# Autodesk Inventor assembly: BrailleTyper
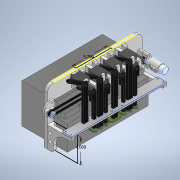
[picture p0: Inventor's stored thumbnail of the model, 180x180]
Saved by Autodesk Inventor 2020.1 (Build 241239000, 239)
## iProperties
Created: 2020-02-22
Part Number: BrailleTyper
Document SubType Name: Assembly
Designer: Dominic
Author: Dominic
## Documents named in this file (21)
- C:\Users\panzi\Dropbox\Projects\Braille\BrailleTyper.iam
- C:\Users\panzi\Dropbox\Projects\Braille\RoughMachine.ipt
- C:\Users\panzi\Dropbox\Projects\Braille\Servo.ipt
- C:\Users\panzi\Dropbox\Projects\Braille\KeyLever.ipt
- C:\Users\panzi\Dropbox\Projects\Braille\ShortBraillePlunger.ipt
- C:\Users\panzi\Dropbox\Projects\Braille\PlungerPlate.ipt
- C:\Users\panzi\Dropbox\Projects\Braille\LongBraillePlunger.ipt
- C:\Users\panzi\Dropbox\Projects\Braille\BigServo.ipt
- C:\Users\panzi\Dropbox\Projects\Braille\NewLinePlunger.ipt
- C:\Users\panzi\Dropbox\Projects\Braille\KeyLeverNewLine.ipt
- C:\Users\panzi\Dropbox\Projects\Braille\Pulley.ipt
- C:\Users\panzi\Dropbox\Projects\Braille\Belt.ipt
- C:\Users\panzi\Dropbox\Projects\Braille\Frame.ipt
- C:\Users\panzi\Dropbox\Projects\Braille\ServoMount.ipt
- C:\Users\panzi\Dropbox\Projects\Braille\ReturnFinger.ipt
- C:\Users\panzi\Dropbox\Projects\Braille\PlungerPlateBracket.ipt
- C:\Users\panzi\Dropbox\Projects\Braille\BigServoMount.ipt
- C:\Users\panzi\Dropbox\Projects\Braille\Tensioner.ipt
- C:\Users\panzi\Dropbox\Projects\Braille\ldo_motor_multiple_configs.ipt
- C:\Users\panzi\Dropbox\Projects\Braille\MotorMount.ipt
- C:\Users\panzi\Dropbox\Projects\Braille\PlungerPlateBracket_MIR1.ipt
## Components (44 placed, 20 different names)
1. RoughMachine:1 — Flush:8, Mate:16, Flush:21, Mate:25, Mate:54, Mate:61, Flush:28, Flush:29
2. Servo:2 — Flush:2, Flush:12, Mate:15, Flush:24, Mate:75, Mate:80, Mate:100, Mate:101, Mate:102
3. Servo:3 — Flush:2, Flush:3, Flush:11, Mate:6, Mate:13, Mate:69, Mate:70, Mate:71
4. Servo:4 — Flush:3, Flush:4, Flush:13, Mate:72, Mate:73, Mate:74, Mate:77, Mate:78
5. Servo:5 — Flush:4, Flush:5, Flush:10, Flush:11, Mate:4, Mate:12, Mate:91, Mate:92, Mate:93
6. Servo:6 — Flush:5, Flush:6, Flush:9, Flush:10, Mate:7, Mate:10, Mate:97, Mate:98, Mate:99
7. Servo:7 — Flush:6, Flush:7, Flush:9, Mate:1, Mate:8, Mate:15, Mate:16, Mate:103, Mate:104, Mate:105
8. Servo:8 — Flush:7, Flush:8, Flush:12, Flush:13, Mate:76, Mate:79, Mate:94, Mate:95, Mate:96
9. KeyLever:1 — Mate:1, Mate:8, Mate:128, Mate:129
10. KeyLever:4 — Mate:4, Mate:12, Mate:89, Mate:127
11. KeyLever:6 — Mate:6, Mate:13, Mate:28, Mate:90
12. KeyLever:7 — Mate:7, Mate:10, Mate:26, Mate:88
13. PlungerPlate:1 — Flush:21, Mate:25, Mate:32, Mate:33, Mate:34, Mate:42, Mate:43, Mate:44, Mate:53, Mate:109, Mate:110, Mate:111, Mate:125, Mate:126, Mate:130
14. ShortBraillePlunger:2 — Mate:26, Mate:32, Mate:88
15. ShortBraillePlunger:3 — Mate:33, Mate:89, Mate:126, Mate:127
16. ShortBraillePlunger:4 — Mate:28, Mate:34, Mate:90
17. LongBraillePlunger:1 — Mate:42, Mate:81, Mate:86
18. LongBraillePlunger:2 — Mate:44, Mate:82, Mate:85
19. LongBraillePlunger:3 — Mate:43, Mate:83, Mate:84
20. BigServo:1 — Flush:24, Mate:55, Mate:56, Mate:112, Mate:113, Mate:114
21. NewLinePlunger:1 — Mate:53, Mate:54, Mate:57, Mate:58
22. KeyLeverNewLine:1 — Mate:55, Mate:56, Mate:57, Mate:58
23. Pulley:1 — Flush:26, Mate:61, Mate:118, Mate:119
24. Pulley:2 — Flush:26, Mate:65, Mate:66, Mate:120
25. Belt:1 — Mate:65, Mate:66, Mate:106, Mate:119, Mate:131
26. Frame:1 — Flush:28, Flush:29, Mate:115, Mate:116, Tangent:1, Mate:117, Tangent:2, Mate:120, Mate:121, Mate:123, Mate:124, Flush:31
27. ServoMount:1 — Mate:69, Mate:70, Mate:71
28. ServoMount:2 — Mate:72, Mate:73, Mate:74
29. KeyLever:8 — Mate:75, Mate:80, Mate:81, Mate:86
30. KeyLever:9 — Mate:76, Mate:79, Mate:82, Mate:85
31. KeyLever:10 — Mate:77, Mate:78, Mate:83, Mate:84
32. ServoMount:3 — Mate:91, Mate:92, Mate:93
33. ServoMount:4 — Mate:94, Mate:95, Mate:96
34. ServoMount:5 — Mate:97, Mate:98, Mate:99
35. ServoMount:6 — Mate:100, Mate:101, Mate:102, Mate:117
36. ServoMount:7 — Mate:103, Mate:104, Mate:105
37. ReturnFinger:1 — Mate:106, Mate:131
38. PlungerPlateBracket:2 — Mate:109, Mate:110, Mate:111
39. BigServoMount:1 — Mate:112, Mate:113, Mate:114, Mate:115
40. Tensioner:1 — Mate:116, Tangent:1, Mate:118, Tangent:2
41. ldo_motor_multiple_configs:1 — Mate:121, Mate:122, Flush:30
42. MotorMount:1 — Mate:122, Mate:123, Mate:124, Flush:30
43. PlungerPlateBracket_MIR1:1 — Mate:125, Flush:31
44. ShortBraillePlunger:5 — Mate:128, Mate:129, Mate:130
## Relationships (109: Mate 88, Flush 19, Tangent 2)
- Flush:2: Servo:2 ↔ Servo:3
- Flush:3: Servo:3 ↔ Servo:4
- Flush:4: Servo:4 ↔ Servo:5
- Flush:5: Servo:5 ↔ Servo:6
- Flush:6: Servo:6 ↔ Servo:7
- Flush:7: Servo:7 ↔ Servo:8
- Flush:8 (-50.8 mm): RoughMachine:1 ↔ Servo:8
- Flush:9: Servo:6 ↔ Servo:7
- Flush:10: Servo:5 ↔ Servo:6
- Flush:11: Servo:3 ↔ Servo:5
- Flush:12: Servo:2 ↔ Servo:8
- Flush:13: Servo:4 ↔ Servo:8
- Mate:1: Servo:7 ↔ KeyLever:1
- Mate:4: Servo:5 ↔ KeyLever:4
- Mate:6: Servo:3 ↔ KeyLever:6
- Mate:7: Servo:6 ↔ KeyLever:7
- Mate:8: Servo:7 ↔ KeyLever:1
- Mate:10: Servo:6 ↔ KeyLever:7
- Mate:12: Servo:5 ↔ KeyLever:4
- Mate:13: Servo:3 ↔ KeyLever:6
- Mate:15 (9.525 mm): Servo:2 ↔ Servo:7
- Mate:16 (69.85 mm): RoughMachine:1 ↔ Servo:7
- Flush:21 (88.9 mm): RoughMachine:1 ↔ PlungerPlate:1
- Mate:25 (9.525 mm): RoughMachine:1 ↔ PlungerPlate:1
- Mate:26: KeyLever:7 ↔ ShortBraillePlunger:2
- Mate:28: KeyLever:6 ↔ ShortBraillePlunger:4
- Mate:32: PlungerPlate:1 ↔ ShortBraillePlunger:2
- Mate:33: PlungerPlate:1 ↔ ShortBraillePlunger:3
- Mate:34: PlungerPlate:1 ↔ ShortBraillePlunger:4
- Mate:42: PlungerPlate:1 ↔ LongBraillePlunger:1
- Mate:43: PlungerPlate:1 ↔ LongBraillePlunger:3
- Mate:44: PlungerPlate:1 ↔ LongBraillePlunger:2
- Flush:24: Servo:2 ↔ BigServo:1
- Mate:53: PlungerPlate:1 ↔ NewLinePlunger:1
- Mate:54: RoughMachine:1 ↔ NewLinePlunger:1
- Mate:55: BigServo:1 ↔ KeyLeverNewLine:1
- Mate:56: BigServo:1 ↔ KeyLeverNewLine:1
- Mate:57: NewLinePlunger:1 ↔ KeyLeverNewLine:1
- Mate:58: NewLinePlunger:1 ↔ KeyLeverNewLine:1
- Flush:26: Pulley:1 ↔ Pulley:2
- Mate:61 (6.35 mm): RoughMachine:1 ↔ Pulley:1
- Mate:65: Pulley:2 ↔ Belt:1
- Mate:66: Pulley:2 ↔ Belt:1
- Flush:28: RoughMachine:1 ↔ Frame:1
- Flush:29: RoughMachine:1 ↔ Frame:1
- Mate:69: Servo:3 ↔ ServoMount:1
- Mate:70: Servo:3 ↔ ServoMount:1
- Mate:71: Servo:3 ↔ ServoMount:1
- Mate:72: Servo:4 ↔ ServoMount:2
- Mate:73: Servo:4 ↔ ServoMount:2
- Mate:74: Servo:4 ↔ ServoMount:2
- Mate:75: Servo:2 ↔ KeyLever:8
- Mate:76: Servo:8 ↔ KeyLever:9
- Mate:77: Servo:4 ↔ KeyLever:10
- Mate:78: Servo:4 ↔ KeyLever:10
- Mate:79: Servo:8 ↔ KeyLever:9
- Mate:80: Servo:2 ↔ KeyLever:8
- Mate:81: LongBraillePlunger:1 ↔ KeyLever:8
- Mate:82: LongBraillePlunger:2 ↔ KeyLever:9
- Mate:83: LongBraillePlunger:3 ↔ KeyLever:10
- Mate:84: LongBraillePlunger:3 ↔ KeyLever:10
- Mate:85: LongBraillePlunger:2 ↔ KeyLever:9
- Mate:86: LongBraillePlunger:1 ↔ KeyLever:8
- Mate:88: KeyLever:7 ↔ ShortBraillePlunger:2
- Mate:89: KeyLever:4 ↔ ShortBraillePlunger:3
- Mate:90: KeyLever:6 ↔ ShortBraillePlunger:4
- Mate:91: Servo:5 ↔ ServoMount:3
- Mate:92: Servo:5 ↔ ServoMount:3
- Mate:93: Servo:5 ↔ ServoMount:3
- Mate:94: Servo:8 ↔ ServoMount:4
- Mate:95: Servo:8 ↔ ServoMount:4
- Mate:96: Servo:8 ↔ ServoMount:4
- Mate:97: Servo:6 ↔ ServoMount:5
- Mate:98: Servo:6 ↔ ServoMount:5
- Mate:99: Servo:6 ↔ ServoMount:5
- Mate:100: Servo:2 ↔ ServoMount:6
- Mate:101: Servo:2 ↔ ServoMount:6
- Mate:102: Servo:2 ↔ ServoMount:6
- Mate:103: Servo:7 ↔ ServoMount:7
- Mate:104: Servo:7 ↔ ServoMount:7
- Mate:105: Servo:7 ↔ ServoMount:7
- Mate:106: Belt:1 ↔ ReturnFinger:1
- Mate:109: PlungerPlate:1 ↔ PlungerPlateBracket:2
- Mate:110: PlungerPlate:1 ↔ PlungerPlateBracket:2
- Mate:111: PlungerPlate:1 ↔ PlungerPlateBracket:2
- Mate:112: BigServo:1 ↔ BigServoMount:1
- Mate:113: BigServo:1 ↔ BigServoMount:1
- Mate:114: BigServo:1 ↔ BigServoMount:1
- Mate:115: Frame:1 ↔ BigServoMount:1
- Mate:116: Frame:1 ↔ Tensioner:1
- Tangent:1: Frame:1 ↔ Tensioner:1
- Mate:117: Frame:1 ↔ ServoMount:6
- Mate:118: Pulley:1 ↔ Tensioner:1
- Tangent:2: Frame:1 ↔ Tensioner:1
- Mate:119: Pulley:1 ↔ Belt:1
- Mate:120: Pulley:2 ↔ Frame:1
- Mate:121: Frame:1 ↔ ldo_motor_multiple_configs:1
- Mate:122: ldo_motor_multiple_configs:1 ↔ MotorMount:1
- Mate:123: Frame:1 ↔ MotorMount:1
- Mate:124: Frame:1 ↔ MotorMount:1
- Flush:30 (15.875 mm): ldo_motor_multiple_configs:1 ↔ MotorMount:1
- Mate:125: PlungerPlate:1 ↔ PlungerPlateBracket_MIR1:1
- Flush:31: Frame:1 ↔ PlungerPlateBracket_MIR1:1
- Mate:126: PlungerPlate:1 ↔ ShortBraillePlunger:3
- Mate:127: KeyLever:4 ↔ ShortBraillePlunger:3
- Mate:128: KeyLever:1 ↔ ShortBraillePlunger:5
- Mate:129: KeyLever:1 ↔ ShortBraillePlunger:5
- Mate:130: PlungerPlate:1 ↔ ShortBraillePlunger:5
- Mate:131: Belt:1 ↔ ReturnFinger:1
